# Autodesk Inventor assembly: AHRS
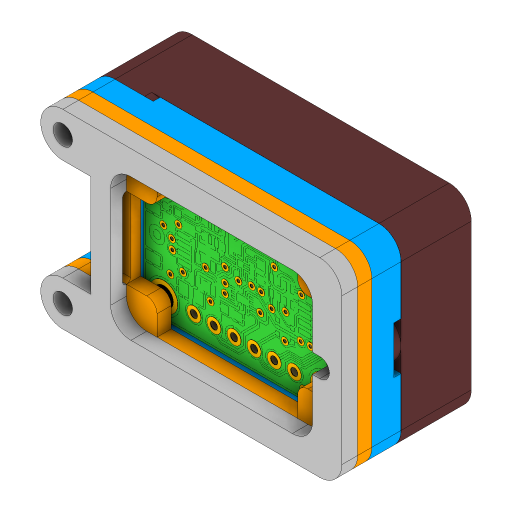
[picture p0: Inventor's stored thumbnail of the model, 512x512]
Saved by Autodesk Inventor 2023 (Build 270158000, 158)
## iProperties
Created: 2022-07-09
Part Number: AHRS
Document SubType Name: Assembly
Designer: Jochen Alt
Author: Jochen Alt
## Documents named in this file (4)
- D:\Projects\Lisbeth\CAD\STL\Accessories\AHRS.iam
- D:\Projects\Lisbeth\CAD\Common\Accessories\Lord Microstrain 3DM-CX5 OEM.ipt
- D:\Projects\Lisbeth\CAD\Common\Accessories\Adafruit LIS3MDL + LSM6DSOX.iam
- D:\Projects\Lisbeth\CAD\Common\Accessories\IMU Holder.ipt
## Components (3 placed, 3 different names)
1. Lord Microstrain IMU OEM:1 — Mate:1, Mate:2
2. Adafruit LIS3MDL + LSM6DSOX:1 [sub-assembly] — Mate:3, Mate:4, Mate:5
3. IMU Holder:1 — Mate:1, Mate:2, Mate:3, Mate:4, Mate:5
## Relationships (5: Mate 5)
- Mate:1: Lord Microstrain IMU OEM:1 ↔ IMU Holder:1
- Mate:2: Lord Microstrain IMU OEM:1 ↔ IMU Holder:1
- Mate:3: Adafruit LIS3MDL + LSM6DSOX:1 ↔ IMU Holder:1
- Mate:4: Adafruit LIS3MDL + LSM6DSOX:1 ↔ IMU Holder:1
- Mate:5: Adafruit LIS3MDL + LSM6DSOX:1 ↔ IMU Holder:1
